# Autodesk Inventor assembly: Overview
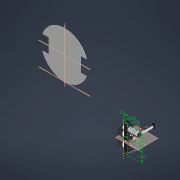
[picture p0: Inventor's stored thumbnail of the model, 180x180]
Saved by Autodesk Inventor 2022 (Build 260153000, 153)
## iProperties
Created: 2021-10-05
Part Number: Overview
Document SubType Name: Assembly
Designer: shiok
Author: shiok
## Documents named in this file (3)
- C:\Users\shiok\Documents\GitHub\Murakumo\inventor\Overview.iam
- C:\Users\shiok\Documents\GitHub\Murakumo\inventor\flame.ipt
- C:\Users\shiok\Documents\GitHub\Murakumo\inventor\Motor.iam
## Components (2 placed, 2 different names)
1. flame:1 — メイト:1, メイト:2, フラッシュ:1
2. Motor:1 [sub-assembly] — メイト:3, メイト:4, メイト:5, メイト:6, 角度:1
## Relationships (10: Mate 8, Angle 1, Flush 1)
- メイト:1 [Mate]: flame:1
- メイト:2 [Mate]: flame:1
- メイト:3 [Mate]: Motor:1
- メイト:4 [Mate]: Motor:1
- メイト:5 [Mate]: Motor:1
- メイト:6 [Mate]: Motor:1
- メイト:7 [Mate]
- メイト:8 [Mate]
- 角度:1 [Angle] (0 deg): Motor:1
- フラッシュ:1 [Flush] (-42.5 mm): flame:1
